# Autodesk Inventor assembly: WithAdapter4Inch60A
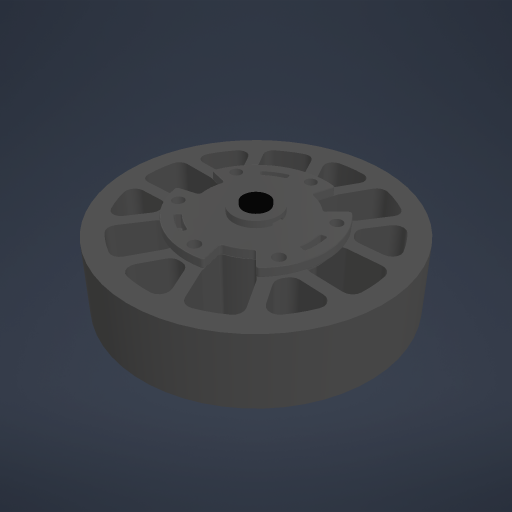
[picture p0: Inventor's stored thumbnail of the model, 512x512]
Saved by Autodesk Inventor 2023 (Build 270158000, 158)
## iProperties
Created: 2022-09-22
Part Number: WithAdapter4Inch60A
Document SubType Name: Assembly
Designer: alex
Author: alex
## Documents named in this file (6)
- C:\Users\alex\Documents\GitHub\4067X_spin_up_cad\WithAdapter4Inch60A.iam
- C:\Users\alex\Documents\GitHub\4067X_spin_up_cad\Library\Motion\Wheels\Flex Wheels\4.000 Flex Wheel\4.000 60A 1.000.ipt
- C:\Users\alex\Documents\GitHub\4067X_spin_up_cad\Library\Motion\Wheels\Flex Wheels\4.000 Flex Wheel.ipt
- C:\Users\alex\Documents\GitHub\4067X_spin_up_cad\Library\Motion\Wheels\Flex Wheels\VersaHub.ipt
- C:\Users\alex\Documents\GitHub\4067X_spin_up_cad\Library\Motion\Wheels\Flex Wheels\VersaHex Adapters .250.ipt
- C:\Users\alex\Documents\GitHub\4067X_spin_up_cad\Library\Motion\Square Insert.ipt
## Components (7 placed, 4 different names)
1. 4.000 60A 1.000:1 — Mate:1, Mate:2, Mate:3, Mate:4, Mate:5, Mate:6
2. VersaHub:1 — Mate:1, Mate:2, Mate:3, Mate:7, Mate:8, Mate:9
3. VersaHub:2 — Mate:4, Mate:5, Mate:6, Mate:10, Mate:11, Mate:12
4. VersaHex Adapters .250:1 — Mate:7, Mate:8, Mate:9, Mate:16, Mate:17, Mate:18
5. VersaHex Adapters .250:2 — Mate:10, Mate:11, Mate:12, Mate:13, Mate:14, Mate:15
6. Square Insert:1 — Mate:13, Mate:14, Mate:15
7. Square Insert:2 — Mate:16, Mate:17, Mate:18
## Relationships (18: Mate 18)
- Mate:1: 4.000 60A 1.000:1 ↔ VersaHub:1
- Mate:2: 4.000 60A 1.000:1 ↔ VersaHub:1
- Mate:3: 4.000 60A 1.000:1 ↔ VersaHub:1
- Mate:4: 4.000 60A 1.000:1 ↔ VersaHub:2
- Mate:5: 4.000 60A 1.000:1 ↔ VersaHub:2
- Mate:6: 4.000 60A 1.000:1 ↔ VersaHub:2
- Mate:7: VersaHub:1 ↔ VersaHex Adapters .250:1
- Mate:8: VersaHub:1 ↔ VersaHex Adapters .250:1
- Mate:9: VersaHub:1 ↔ VersaHex Adapters .250:1
- Mate:10: VersaHub:2 ↔ VersaHex Adapters .250:2
- Mate:11: VersaHub:2 ↔ VersaHex Adapters .250:2
- Mate:12: VersaHub:2 ↔ VersaHex Adapters .250:2
- Mate:13: VersaHex Adapters .250:2 ↔ Square Insert:1
- Mate:14: VersaHex Adapters .250:2 ↔ Square Insert:1
- Mate:15: VersaHex Adapters .250:2 ↔ Square Insert:1
- Mate:16: VersaHex Adapters .250:1 ↔ Square Insert:2
- Mate:17: VersaHex Adapters .250:1 ↔ Square Insert:2
- Mate:18: VersaHex Adapters .250:1 ↔ Square Insert:2
